# Autodesk Inventor assembly: robotface
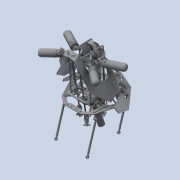
[picture p0: Inventor's stored thumbnail of the model, 180x180]
Saved by Autodesk Inventor 2020 (Build 240168000, 168)
## iProperties
Created: 2021-06-30
Part Number: robotface
Document SubType Name: Assembly
Designer: valer
Author: valer
## Documents named in this file (49)
- C:\Users\Val\Desktop\drummingrobot\design\robotface\robotface.iam
- C:\Users\Val\Desktop\drummingrobot\design\robotface\robotface-final.ipt
- C:\Users\Val\Desktop\drummingrobot\src\parts\external\HingedThreadedStandoffPart2.ipt
- C:\Users\Val\Desktop\drummingrobot\src\parts\external\HingedThreadedStandoffPart1.ipt
- C:\Users\Val\Desktop\drummingrobot\design\robotface\TongueMount.ipt
- C:\Users\Val\Desktop\drummingrobot\design\robotface\HeadMount.ipt
- C:\Users\Val\Desktop\drummingrobot\design\robotface\LinearBearing-1612-0612-0035.ipt
- C:\Users\Val\Desktop\drummingrobot\design\robotface\ClampingHub1301-0016-0012.ipt
- C:\Users\Val\Desktop\drummingrobot\design\robotface\UJoint6D\UJoint6D-Body-4003-1006-1006.ipt
- C:\Users\Val\Desktop\drummingrobot\design\robotface\UJoint6D\UJoint6D-CenterDrive-4003-1006-1006.ipt
- C:\Users\Val\Desktop\drummingrobot\design\robotface\UJoint6D\UJoint6D-Screw.ipt
- C:\Users\Val\Desktop\drummingrobot\design\robotface\SetScrewLiteHub-1308-0016-0006.ipt
- C:\Users\Val\Desktop\drummingrobot\design\robotface\ShaftD6-Short-2101-0006-0020.ipt
- C:\Users\Val\Desktop\drummingrobot\design\robotface\SetScrewHub-1300-0016-1006.ipt
- C:\Users\Val\Desktop\drummingrobot\design\robotface\ShaftD6Female-632Female.ipt
- C:\Users\Val\Desktop\drummingrobot\design\robotface\ShaftD6-2101-0006-0160.ipt
- C:\Users\Val\Desktop\drummingrobot\design\robotface\HeadTongueMount.ipt
- C:\Users\Val\Desktop\drummingrobot\design\robotface\ShaftD6-2100-0006-0250.ipt
- C:\Users\Val\Desktop\drummingrobot\design\robotface\Rod4mm.ipt
- C:\Users\Val\Desktop\drummingrobot\design\robotface\NoseBentBar.ipt
- C:\Users\Val\Desktop\drummingrobot\design\robotface\HeadTopConnector.ipt
- C:\Users\Val\Desktop\drummingrobot\design\robotface\GoTube-4103-0032-0120.ipt
- C:\Users\Val\Desktop\drummingrobot\design\robotface\UJointSq-4005-0016-0001\4005-0016-0001 Ball.ipt
- C:\Users\Val\Desktop\drummingrobot\design\robotface\UJointSq-4005-0016-0001\4005-0016-0001 Outer Shell.ipt
- C:\Users\Val\Desktop\drummingrobot\design\robotface\7417N62_INTERNALLY THREADED CONNECTING ROD.ipt
- C:\Users\Val\Desktop\drummingrobot\design\robotface\RodEndFixed-2434K495_CORROSION-RESISTANT FULLY THREADED ROD END BOLT.ipt
- C:\Users\Val\Desktop\drummingrobot\design\robotface\StandoffM4-1501-0006-0420.ipt
- C:\Users\Val\Desktop\drummingrobot\design\robotface\StandoffM4-1501-0006-0340.ipt
- C:\Users\Val\Desktop\drummingrobot\src\parts\external\Arducam.ipt
- C:\Users\Val\Desktop\drummingrobot\src\parts\external\ArducamHat.ipt
- C:\Users\Val\Desktop\drummingrobot\design\robotface\HeadEyeMount.ipt
- C:\Users\Val\Desktop\drummingrobot\design\robotface\M3-Standoff-30mm.ipt
- C:\Users\Val\Desktop\drummingrobot\design\robotface\M5-Standoff-32mm.ipt
- C:\Users\Val\Desktop\drummingrobot\src\parts\external\ArducamMirror.ipt
- C:\Users\Val\Desktop\drummingrobot\design\robotface\M1-Standoff-20mm.ipt
- C:\Users\Val\Desktop\drummingrobot\design\robotface\NoseInsideConnector.ipt
- C:\Users\Val\Desktop\drummingrobot\design\robotface\Part2^3mm U-Joint.ipt
- C:\Users\Val\Desktop\drummingrobot\design\robotface\Part1^3mm U-Joint.ipt
- C:\Users\Val\Desktop\drummingrobot\design\robotface\NoseCover.ipt
- C:\Users\Val\Desktop\drummingrobot\design\robotface\NoseCoverSmall.ipt
- C:\Users\Val\Desktop\drummingrobot\design\robotface\IRLed-FY-4006.ipt
- C:\Users\Val\Desktop\drummingrobot\design\robotface\BackEyeMountLeft.ipt
- C:\Users\Val\Desktop\drummingrobot\design\robotface\BackEyeMountRight.ipt
- C:\Users\Val\Desktop\drummingrobot\design\robotface\ShaftClamp6-6058N14.ipt
- C:\Users\Val\Desktop\drummingrobot\design\robotface\MuzzleHeadMount.ipt
- C:\Users\Val\Desktop\drummingrobot\design\robotface\ShaftD6-2100-0006-0200.ipt
- C:\Users\Val\Desktop\drummingrobot\design\robotface\MuzzleHeadConnector.ipt
- C:\Users\Val\Desktop\drummingrobot\src\parts\VacuumTubeHolder.iam
- C:\Users\Val\Desktop\drummingrobot\src\parts\FaceTubeConnector.ipt
## Components (180 placed, 48 different names)
1. robotface-final:1 — Mate:7, Mate:8, Mate:9, Mate:10, Mate:11, Mate:12, Angle:3, Mate:18, Mate:19, Mate:20, Mate:25, Mate:26, Mate:90, Mate:91, Mate:92, Mate:93, Angle:18, Angle:20, Mate:132, Mate:133, Angle:28, Mate:189, Mate:190, Angle:35, Angle:36, Mate:205, Angle:41, Mate:242, Mate:244, Mate:245, Mate:246, Mate:247, Mate:248, Mate:249, Mate:250, Mate:251, Mate:254, Mate:255, Angle:47, Mate:277, Mate:278, Mate:282, Mate:368, Mate:369, Angle:58, Mate:380, Mate:381, Mate:382, Mate:383, Mate:386, Mate:387, Mate:389, Mate:404, Mate:405, Mate:414, Mate:415, Mate:416, Mate:417, Mate:418, Mate:419, Mate:463, Mate:465, Mate:469, Mate:474
2. HingedThreadedStandoffPart2:1 — Mate:1, Mate:2, Flush:1, Angle:4, Mate:284
3. HingedThreadedStandoffPart1:1 — Mate:1, Mate:2, Mate:7, Mate:8
4. HingedThreadedStandoffPart2:2 — Mate:3, Mate:4, Mate:9, Mate:10
5. HingedThreadedStandoffPart1:2 — Mate:3, Mate:4, Flush:1
6. HingedThreadedStandoffPart2:3 — Mate:5, Mate:6, Mate:11, Mate:12, Angle:3, Mate:60, Mate:61
7. HingedThreadedStandoffPart1:3 — Mate:5, Mate:6, Angle:4
8. HingedThreadedStandoffPart2:4 — Mate:18, Mate:19, Mate:20, Mate:21, Mate:22
9. HingedThreadedStandoffPart1:4 — Mate:21, Mate:22, Mate:89
10. HingedThreadedStandoffPart2:5 — Mate:25, Mate:26
11. HingedThreadedStandoffPart1:5 — Mate:85, Mate:86
12. TongueMount:2 — Mate:278, Mate:281, Mate:283, Mate:284, Flush:24
13. HeadMount:1 — Mate:110, Mate:111, Mate:112, Flush:12, Mate:210, Mate:211, Mate:212, Mate:213, Mate:214, Mate:215, Mate:216, Mate:217, Mate:342, Mate:345, Mate:346, Mate:347, Mate:392, Mate:393, Mate:394, Mate:398, Mate:399, Mate:400
14. LinearBearing-1612-0612-0035:1 — Mate:299, Mate:300, Flush:25
15. ClampingHub1301-0016-0012:1 — Mate:115, Mate:282, Mate:300, Flush:25
16. ShaftD6-2100-0006-0250:1 — Mate:298, Angle:52, Flush:23, Angle:54, Mate:299, Mate:311, Angle:55, Flush:26
17. SetScrewLiteHub-1308-0016-0006:1 — Mate:65, Mate:67, Mate:281, Angle:53, Flush:24
18. HingedThreadedStandoffPart2:6 — Mate:60, Mate:61, Mate:283
19. ShaftD6-Short-2101-0006-0020:1 — Mate:65, Mate:67, Angle:51, Mate:297, Flush:22
20. ShaftD6-2101-0006-0160:2 — Mate:87, Angle:16
21. ShaftD6-2101-0006-0160:3
22. SetScrewHub-1300-0016-1006:1 — Mate:114
23. SetScrewHub-1300-0016-1006:2 — Mate:113
24. ShaftD6Female-632Female:1 — Mate:85, Mate:86
25. ShaftD6Female-632Female:2 — Mate:87, Mate:89, Angle:16
26. HingedThreadedStandoffPart2:9 — Mate:92, Mate:93, Mate:96, Mate:97
27. HingedThreadedStandoffPart2:10 — Mate:90, Mate:91, Mate:94, Mate:95
28. HingedThreadedStandoffPart2:11 — Mate:94, Mate:95, Mate:98, Mate:99
29. HingedThreadedStandoffPart2:12 — Mate:96, Mate:97, Mate:100, Mate:101
30. ShaftD6Female-632Female:3 — Mate:98, Mate:99, Mate:102, Angle:17, Mate:103, Angle:18
31. ShaftD6Female-632Female:4 — Mate:100, Mate:101, Mate:104, Angle:19, Angle:20, Mate:105
32. ShaftD6-2101-0006-0160:4 — Mate:102, Angle:17, Mate:103, Mate:106, Angle:21
33. ShaftD6-2101-0006-0160:5 — Mate:104, Angle:19, Mate:105, Mate:107, Angle:22
34. SetScrewHub-1300-0016-1006:3 — Mate:106, Angle:21, Mate:116
35. SetScrewHub-1300-0016-1006:4 — Mate:107, Angle:22, Mate:117
36. HeadTongueMount:1 — Mate:110, Mate:111, Mate:112, Mate:113, Mate:114, Mate:115, Mate:116, Mate:117, Mate:204, Angle:39, Flush:15, Angle:54, Mate:431
37. Rod4mm:1 — Mate:132
38. Rod4mm:2 — Mate:133
39. SetScrewLiteHub-1308-0016-0006:2 — Mate:151, Flush:5, Mate:153, Angle:26, Mate:242, Mate:370, Mate:371
40. UJoint6D-Body-4003-1006-1006:5 — Mate:154, Angle:27, Flush:6, Angle:28
41. UJoint6D-CenterDrive-4003-1006-1006:3
42. UJoint6D-Screw:11
43. UJoint6D-Body-4003-1006-1006:6 — Mate:152, Angle:25, Mate:153, Angle:26
44. UJoint6D-Screw:12
45. UJoint6D-Screw:13
46. UJoint6D-Screw:14
47. ShaftD6-Short-2101-0006-0020:2 — Mate:151, Flush:5, Mate:152, Angle:25
48. ShaftD6-2100-0006-0250:2 — Mate:154, Angle:27, Flush:6, Mate:167, Angle:29, Flush:7
49. UJoint6D-Body-4003-1006-1006:7 — Mate:184, Angle:32, Flush:9, Mate:185, Angle:38
50. UJoint6D-CenterDrive-4003-1006-1006:4
51. UJoint6D-Screw:15
52. UJoint6D-Body-4003-1006-1006:8 — Mate:167, Angle:29, Flush:7
53. UJoint6D-Screw:16
54. UJoint6D-Screw:17
55. UJoint6D-Screw:18
56. SetScrewLiteHub-1308-0016-0006:3 — Mate:185, Mate:186, Angle:38
57. ShaftD6-Short-2101-0006-0020:3 — Mate:184, Angle:32, Flush:9, Mate:186
58. ShaftD6-Short-2101-0006-0020:4 — Mate:312, Angle:56, Flush:27, Mate:313, Flush:28
59. NoseBentBar:1 — Mate:189, Angle:36, Flush:13, Flush:14
60. NoseBentBar:2 — Mate:190, Angle:35, Flush:13
61. HeadTopConnector:1 — Flush:12, Flush:14
62. GoTube-4103-0032-0120:1 — Mate:201, Mate:202, Mate:203
63. 4005-0016-0001 Ball:1 — Mate:197, Mate:198, Mate:199, Mate:200
64. 4005-0016-0001 Outer Shell:1 — Mate:197, Mate:198, Mate:204, Angle:39, Flush:15, Mate:205
65. 4005-0016-0001 Outer Shell:2 — Mate:199, Mate:200, Mate:201, Mate:202, Mate:203
66. 7417N62_INTERNALLY THREADED CONNECTING ROD:1 — Mate:218, Mate:219, Mate:220, Mate:222
67. RodEndFixed-2434K495_CORROSION-RESISTANT FULLY THREADED ROD END BOLT:1 — Mate:210, Mate:211, Angle:40, Angle:41, Angle:42, Mate:221, Mate:223
68. RodEndFixed-2434K495_CORROSION-RESISTANT FULLY THREADED ROD END BOLT:2 — Mate:212, Mate:213, Angle:40, Mate:228, Mate:229
69. RodEndFixed-2434K495_CORROSION-RESISTANT FULLY THREADED ROD END BOLT:3 — Mate:214, Mate:215, Angle:42, Angle:43, Mate:240, Mate:241
70. RodEndFixed-2434K495_CORROSION-RESISTANT FULLY THREADED ROD END BOLT:4 — Mate:216, Mate:217, Angle:43, Mate:234, Mate:235
71. RodEndFixed-2434K495_CORROSION-RESISTANT FULLY THREADED ROD END BOLT:5 — Mate:218, Mate:220, Mate:221, Mate:223
72. RodEndFixed-2434K495_CORROSION-RESISTANT FULLY THREADED ROD END BOLT:6 — Mate:219, Mate:222, Angle:44, Angle:46
73. 7417N62_INTERNALLY THREADED CONNECTING ROD:2
74. RodEndFixed-2434K495_CORROSION-RESISTANT FULLY THREADED ROD END BOLT:7 — Mate:228, Mate:229
75. RodEndFixed-2434K495_CORROSION-RESISTANT FULLY THREADED ROD END BOLT:8 — Angle:44, Angle:45
76. 7417N62_INTERNALLY THREADED CONNECTING ROD:3
77. RodEndFixed-2434K495_CORROSION-RESISTANT FULLY THREADED ROD END BOLT:9 — Mate:234, Mate:235
78. RodEndFixed-2434K495_CORROSION-RESISTANT FULLY THREADED ROD END BOLT:10 — Angle:45
79. 7417N62_INTERNALLY THREADED CONNECTING ROD:4
80. RodEndFixed-2434K495_CORROSION-RESISTANT FULLY THREADED ROD END BOLT:11 — Mate:240, Mate:241
81. RodEndFixed-2434K495_CORROSION-RESISTANT FULLY THREADED ROD END BOLT:12 — Angle:46
82. StandoffM4-1501-0006-0420:1 — Mate:244, Mate:245
83. StandoffM4-1501-0006-0420:2 — Mate:246, Mate:247
84. StandoffM4-1501-0006-0340:1 — Mate:248, Mate:249
85. StandoffM4-1501-0006-0340:2 — Mate:250, Mate:251
86. HingedThreadedStandoffPart2:13 — Mate:256, Mate:257
87. HingedThreadedStandoffPart1:6 — Mate:254, Mate:255, Angle:47
88. ShaftD6Female-632Female:5 — Mate:256, Mate:257, Mate:273, Angle:50, Mate:274
89. ShaftD6-2100-0006-0250:3 — Mate:273, Angle:50, Mate:274
90. UJoint6D-Body-4003-1006-1006:9
91. UJoint6D-CenterDrive-4003-1006-1006:5
92. UJoint6D-Screw:19
93. UJoint6D-Body-4003-1006-1006:10
94. UJoint6D-Screw:20
95. UJoint6D-Screw:21
96. UJoint6D-Screw:22
97. SetScrewLiteHub-1308-0016-0006:5
98. ShaftD6-Short-2101-0006-0020:5
99. ArducamHat:1 — Mate:314, Mate:316, Mate:317, Mate:318, Mate:319
100. Arducam:2 — Mate:350, Mate:351, Mate:352, Mate:354, Mate:356, Mate:364, Mate:390
101. HeadEyeMount:1 — Mate:277, Mate:315, Mate:320, Mate:341, Mate:343, Mate:344, Mate:348, Mate:349, Mate:350, Mate:351, Mate:353, Mate:355, Mate:357, Mate:359, Mate:360, Mate:362, Mate:365, Mate:367
102. UJoint6D-Body-4003-1006-1006:11 — Mate:298, Angle:52, Flush:23
103. UJoint6D-CenterDrive-4003-1006-1006:6
104. UJoint6D-Screw:23
105. UJoint6D-Body-4003-1006-1006:12 — Angle:51, Mate:297, Flush:22, Angle:53
106. UJoint6D-Screw:24
107. UJoint6D-Screw:25
108. UJoint6D-Screw:26
109. UJoint6D-Body-4003-1006-1006:13 — Mate:312, Angle:56, Flush:27, Angle:57
110. UJoint6D-CenterDrive-4003-1006-1006:7
111. UJoint6D-Body-4003-1006-1006:14 — Mate:311, Angle:55, Flush:26
112. UJoint6D-Screw:27
113. UJoint6D-Screw:28
114. UJoint6D-Screw:29
115. SetScrewLiteHub-1308-0016-0006:6 — Mate:313, Angle:57, Flush:28
116. M3-Standoff-30mm:1 — Mate:314, Mate:315, Mate:316
117. M3-Standoff-30mm:2 — Mate:317, Mate:318
118. M3-Standoff-30mm:3 — Mate:319, Mate:320
119. M5-Standoff-32mm:1 — Mate:341, Mate:342, Mate:343
120. M5-Standoff-32mm:2 — Mate:344, Mate:345
121. M5-Standoff-32mm:3 — Mate:346, Mate:349
122. M5-Standoff-32mm:4 — Mate:347, Mate:348
123. ArducamMirror:1 — Mate:358, Mate:361, Mate:363, Mate:366, Mate:391
124. M1-Standoff-20mm:1 — Mate:352, Mate:353
125. M1-Standoff-20mm:2 — Mate:354, Mate:355, Mate:364
126. M1-Standoff-20mm:3 — Mate:356, Mate:357
127. M1-Standoff-20mm:4 — Mate:358, Mate:359, Mate:360
128. M1-Standoff-20mm:5 — Mate:361, Mate:362, Mate:363, Mate:365
129. M1-Standoff-20mm:6 — Mate:366, Mate:367
130. NoseInsideConnector:1 — Mate:368, Mate:369, Angle:58, Mate:370, Mate:371, Mate:384, Mate:385
131. Part2^3mm U-Joint:1 — Mate:372, Mate:373, Mate:374, Mate:375
132. Part1^3mm U-Joint:1 — Mate:372, Mate:373, Mate:385
133. Part1^3mm U-Joint:2 — Mate:374, Mate:375, Mate:380, Mate:381
134. Part2^3mm U-Joint:2
135. Part1^3mm U-Joint:3 — Mate:384
136. Part1^3mm U-Joint:4 — Mate:382, Mate:383
137. NoseCover:1 — Mate:386, Mate:387, Flush:29, Mate:388
138. NoseCoverSmall:1 — Flush:29, Mate:388, Mate:389
139. IRLed-FY-4006:1 — Mate:391
140. IRLed-FY-4006:2 — Mate:390
141. IRLed-FY-4006:3 — Mate:395, Mate:396, Mate:397
142. BackEyeMountRight:1 — Mate:398, Mate:399, Mate:400, Mate:401, Mate:402, Mate:403
143. BackEyeMountLeft:1 — Mate:392, Mate:393, Mate:394, Mate:395, Mate:396, Mate:397
144. IRLed-FY-4006:4 — Mate:401, Mate:402, Mate:403
145. ShaftD6-2100-0006-0200:1 — Mate:432, Mate:436
146. ShaftClamp6-6058N14:1 — Mate:404, Mate:405
147. ShaftD6-2100-0006-0200:2 — Mate:441, Mate:443, Mate:458
148. ShaftClamp6-6058N14:2 — Mate:464
149. ShaftD6-2100-0006-0200:3 — Mate:445, Mate:447, Mate:466
150. ShaftClamp6-6058N14:3
151. ShaftClamp6-6058N14:4 — Mate:414, Mate:415
152. ShaftClamp6-6058N14:5 — Mate:416, Mate:417
153. ShaftD6-2100-0006-0200:4 — Mate:437, Mate:439
154. ShaftClamp6-6058N14:6 — Mate:418, Mate:419
155. ShaftD6-2100-0006-0200:5 — Mate:449, Mate:451, Mate:475
156. ShaftClamp6-6058N14:7 — Mate:476
157. ShaftD6-2100-0006-0200:6 — Mate:453, Mate:455, Mate:470
158. ShaftClamp6-6058N14:8 — Mate:471
159. MuzzleHeadMount:1 — Mate:428, Mate:429, Mate:430, Mate:434, Mate:435, Mate:438, Mate:440, Mate:442, Mate:444, Mate:446, Mate:448, Mate:450, Mate:452, Mate:454, Mate:456
160. MuzzleHeadConnector:1 — Mate:428, Mate:429, Mate:430, Mate:431
161. ShaftClamp6-6058N14:9 — Mate:432, Mate:434
162. ShaftClamp6-6058N14:10 — Mate:435, Mate:436
163. ShaftClamp6-6058N14:12 — Mate:437, Mate:438
164. ShaftClamp6-6058N14:13 — Mate:439, Mate:440
165. ShaftClamp6-6058N14:14 — Mate:441, Mate:442
166. ShaftClamp6-6058N14:15 — Mate:443, Mate:444
167. ShaftClamp6-6058N14:16 — Mate:445, Mate:446
168. ShaftClamp6-6058N14:17 — Mate:447, Mate:448
169. ShaftClamp6-6058N14:18 — Mate:449, Mate:450
170. ShaftClamp6-6058N14:19 — Mate:451, Mate:452
171. ShaftClamp6-6058N14:20 — Mate:453, Mate:454
172. ShaftClamp6-6058N14:21 — Mate:455, Mate:456
173. VacuumTubeHolder:1 [sub-assembly] — Mate:467, Mate:468
174. VacuumTubeHolder:2 [sub-assembly] — Mate:461, Mate:462
175. VacuumTubeHolder:3 [sub-assembly] — Mate:477, Mate:478
176. VacuumTubeHolder:4 [sub-assembly] — Mate:472, Mate:473
177. BackSideConnector:1 — Mate:458, Mate:461, Mate:462, Mate:463, Mate:464
178. BackSideConnector:2 — Mate:465, Mate:466, Mate:467, Mate:468
179. BackSideConnector:3 — Mate:469, Mate:470, Mate:471, Mate:472, Mate:473
180. BackSideConnector:4 — Mate:474, Mate:475, Mate:476, Mate:477, Mate:478
## Relationships (411: Mate 342, Angle 45, Flush 24)
- Mate:1: HingedThreadedStandoffPart2:1 ↔ HingedThreadedStandoffPart1:1
- Mate:2: HingedThreadedStandoffPart2:1 ↔ HingedThreadedStandoffPart1:1
- Mate:3: HingedThreadedStandoffPart2:2 ↔ HingedThreadedStandoffPart1:2
- Mate:4: HingedThreadedStandoffPart2:2 ↔ HingedThreadedStandoffPart1:2
- Mate:5: HingedThreadedStandoffPart2:3 ↔ HingedThreadedStandoffPart1:3
- Mate:6: HingedThreadedStandoffPart2:3 ↔ HingedThreadedStandoffPart1:3
- Mate:7: robotface-final:1 ↔ HingedThreadedStandoffPart1:1
- Mate:8: robotface-final:1 ↔ HingedThreadedStandoffPart1:1
- Mate:9: robotface-final:1 ↔ HingedThreadedStandoffPart2:2
- Mate:10: robotface-final:1 ↔ HingedThreadedStandoffPart2:2
- Mate:11: robotface-final:1 ↔ HingedThreadedStandoffPart2:3
- Mate:12: robotface-final:1 ↔ HingedThreadedStandoffPart2:3
- Angle:3 (0 deg): robotface-final:1 ↔ HingedThreadedStandoffPart2:3
- Mate:18: robotface-final:1 ↔ HingedThreadedStandoffPart2:4
- Mate:19: robotface-final:1 ↔ HingedThreadedStandoffPart2:4
- Mate:20: robotface-final:1 ↔ HingedThreadedStandoffPart2:4
- Mate:21: HingedThreadedStandoffPart2:4 ↔ HingedThreadedStandoffPart1:4
- Mate:22: HingedThreadedStandoffPart2:4 ↔ HingedThreadedStandoffPart1:4
- [Mate]: HingedThreadedStandoffPart2:5 ↔ HingedThreadedStandoffPart1:5
- [Mate]: HingedThreadedStandoffPart2:5 ↔ HingedThreadedStandoffPart1:5
- Mate:25: robotface-final:1 ↔ HingedThreadedStandoffPart2:5
- Mate:26: robotface-final:1 ↔ HingedThreadedStandoffPart2:5
- Flush:1: HingedThreadedStandoffPart2:1 ↔ HingedThreadedStandoffPart1:2
- Angle:4 (0 deg): HingedThreadedStandoffPart2:1 ↔ HingedThreadedStandoffPart1:3
- Mate:60: HingedThreadedStandoffPart2:3 ↔ HingedThreadedStandoffPart2:6
- Mate:61: HingedThreadedStandoffPart2:3 ↔ HingedThreadedStandoffPart2:6
- Mate:65: SetScrewLiteHub-1308-0016-0006:1 ↔ ShaftD6-Short-2101-0006-0020:1
- Mate:67 (-7 mm): SetScrewLiteHub-1308-0016-0006:1 ↔ ShaftD6-Short-2101-0006-0020:1
- [Mate]: HingedThreadedStandoffPart1:4 ↔ ShaftD6-2101-0006-0160:2
- [Angle] (0 deg): HeadMount:1 ↔ ShaftD6-2101-0006-0160:2
- [Mate]: HingedThreadedStandoffPart1:5 ↔ ShaftD6-2101-0006-0160:3
- [Angle] (0 deg): HeadMount:1 ↔ ShaftD6-2101-0006-0160:3
- [Mate]: ShaftD6-2101-0006-0160:2 ↔ SetScrewHub-1300-0016-1006:1
- [Mate]: ShaftD6-2101-0006-0160:3 ↔ SetScrewHub-1300-0016-1006:2
- [Angle] (0 deg): ShaftD6-2101-0006-0160:2 ↔ SetScrewHub-1300-0016-1006:1
- [Angle] (0 deg): ShaftD6-2101-0006-0160:3 ↔ SetScrewHub-1300-0016-1006:2
- [Angle] (0 deg): robotface-final:1 ↔ ShaftD6-2101-0006-0160:2
- [Angle] (0 deg): robotface-final:1 ↔ ShaftD6-2101-0006-0160:3
- [Mate]: ShaftD6-2101-0006-0160:3 ↔ ShaftD6Female-632Female:1
- [Angle] (0 deg): ShaftD6-2101-0006-0160:3 ↔ ShaftD6Female-632Female:1
- [Mate]: ShaftD6-2101-0006-0160:3 ↔ ShaftD6Female-632Female:1
- Mate:85: HingedThreadedStandoffPart1:5 ↔ ShaftD6Female-632Female:1
- Mate:86: HingedThreadedStandoffPart1:5 ↔ ShaftD6Female-632Female:1
- Mate:87: ShaftD6-2101-0006-0160:2 ↔ ShaftD6Female-632Female:2
- Mate:89: HingedThreadedStandoffPart1:4 ↔ ShaftD6Female-632Female:2
- Angle:16 (0 deg): ShaftD6-2101-0006-0160:2 ↔ ShaftD6Female-632Female:2
- Mate:90: robotface-final:1 ↔ HingedThreadedStandoffPart2:10
- Mate:91: robotface-final:1 ↔ HingedThreadedStandoffPart2:10
- Mate:92: robotface-final:1 ↔ HingedThreadedStandoffPart2:9
- Mate:93: robotface-final:1 ↔ HingedThreadedStandoffPart2:9
- Mate:94: HingedThreadedStandoffPart2:10 ↔ HingedThreadedStandoffPart2:11
- Mate:95: HingedThreadedStandoffPart2:10 ↔ HingedThreadedStandoffPart2:11
- Mate:96: HingedThreadedStandoffPart2:9 ↔ HingedThreadedStandoffPart2:12
- Mate:97: HingedThreadedStandoffPart2:9 ↔ HingedThreadedStandoffPart2:12
- Mate:98: HingedThreadedStandoffPart2:11 ↔ ShaftD6Female-632Female:3
- Mate:99: HingedThreadedStandoffPart2:11 ↔ ShaftD6Female-632Female:3
- Mate:100: HingedThreadedStandoffPart2:12 ↔ ShaftD6Female-632Female:4
- Mate:101: HingedThreadedStandoffPart2:12 ↔ ShaftD6Female-632Female:4
- Mate:102: ShaftD6Female-632Female:3 ↔ ShaftD6-2101-0006-0160:4
- Angle:17 (0 deg): ShaftD6Female-632Female:3 ↔ ShaftD6-2101-0006-0160:4
- Mate:103: ShaftD6Female-632Female:3 ↔ ShaftD6-2101-0006-0160:4
- Angle:18 (180 deg): robotface-final:1 ↔ ShaftD6Female-632Female:3
- Mate:104: ShaftD6Female-632Female:4 ↔ ShaftD6-2101-0006-0160:5
- Angle:19 (0 deg): ShaftD6Female-632Female:4 ↔ ShaftD6-2101-0006-0160:5
- Angle:20 (180 deg): robotface-final:1 ↔ ShaftD6Female-632Female:4
- Mate:105: ShaftD6Female-632Female:4 ↔ ShaftD6-2101-0006-0160:5
- Mate:106: ShaftD6-2101-0006-0160:4 ↔ SetScrewHub-1300-0016-1006:3
- Angle:21 (180 deg): ShaftD6-2101-0006-0160:4 ↔ SetScrewHub-1300-0016-1006:3
- Mate:107: ShaftD6-2101-0006-0160:5 ↔ SetScrewHub-1300-0016-1006:4
- Angle:22 (180 deg): ShaftD6-2101-0006-0160:5 ↔ SetScrewHub-1300-0016-1006:4
- Mate:110: HeadMount:1 ↔ HeadTongueMount:1
- Mate:111: HeadMount:1 ↔ HeadTongueMount:1
- Mate:112: HeadMount:1 ↔ HeadTongueMount:1
- Mate:113: SetScrewHub-1300-0016-1006:2 ↔ HeadTongueMount:1
- Mate:114: SetScrewHub-1300-0016-1006:1 ↔ HeadTongueMount:1
- Mate:115: ClampingHub1301-0016-0012:1 ↔ HeadTongueMount:1
- Mate:116: SetScrewHub-1300-0016-1006:3 ↔ HeadTongueMount:1
- Mate:117: SetScrewHub-1300-0016-1006:4 ↔ HeadTongueMount:1
- Mate:132: robotface-final:1 ↔ Rod4mm:1
- Mate:133: robotface-final:1 ↔ Rod4mm:2
- [Mate]: UJoint6D-CenterDrive-4003-1006-1006:3 ↔ UJoint6D-Body-4003-1006-1006:6
- [Mate]: UJoint6D-CenterDrive-4003-1006-1006:3 ↔ UJoint6D-Body-4003-1006-1006:6
- [Mate]: UJoint6D-Body-4003-1006-1006:5 ↔ UJoint6D-CenterDrive-4003-1006-1006:3
- [Mate]: UJoint6D-Body-4003-1006-1006:5 ↔ UJoint6D-CenterDrive-4003-1006-1006:3
- [Mate]: UJoint6D-Body-4003-1006-1006:5 ↔ UJoint6D-Screw:11
- [Mate]: UJoint6D-Body-4003-1006-1006:5 ↔ UJoint6D-Screw:11
- [Mate]: UJoint6D-Body-4003-1006-1006:5 ↔ UJoint6D-Screw:13
- [Mate]: UJoint6D-Body-4003-1006-1006:5 ↔ UJoint6D-Screw:13
- [Mate]: UJoint6D-Body-4003-1006-1006:6 ↔ UJoint6D-Screw:12
- [Mate]: UJoint6D-Body-4003-1006-1006:6 ↔ UJoint6D-Screw:12
- [Mate]: UJoint6D-Body-4003-1006-1006:6 ↔ UJoint6D-Screw:14
- [Mate]: UJoint6D-Body-4003-1006-1006:6 ↔ UJoint6D-Screw:14
- Mate:151: SetScrewLiteHub-1308-0016-0006:2 ↔ ShaftD6-Short-2101-0006-0020:2
- Flush:5: SetScrewLiteHub-1308-0016-0006:2 ↔ ShaftD6-Short-2101-0006-0020:2
- Mate:152: UJoint6D-Body-4003-1006-1006:6 ↔ ShaftD6-Short-2101-0006-0020:2
- Angle:25 (180 deg): UJoint6D-Body-4003-1006-1006:6 ↔ ShaftD6-Short-2101-0006-0020:2
- Mate:153: SetScrewLiteHub-1308-0016-0006:2 ↔ UJoint6D-Body-4003-1006-1006:6
- Angle:26 (0 deg): SetScrewLiteHub-1308-0016-0006:2 ↔ UJoint6D-Body-4003-1006-1006:6
- Mate:154: UJoint6D-Body-4003-1006-1006:5 ↔ ShaftD6-2100-0006-0250:2
- Angle:27 (180 deg): UJoint6D-Body-4003-1006-1006:5 ↔ ShaftD6-2100-0006-0250:2
- Flush:6: UJoint6D-Body-4003-1006-1006:5 ↔ ShaftD6-2100-0006-0250:2
- Angle:28 (0 deg): robotface-final:1 ↔ UJoint6D-Body-4003-1006-1006:5
- [Mate]: UJoint6D-CenterDrive-4003-1006-1006:4 ↔ UJoint6D-Body-4003-1006-1006:8
- [Mate]: UJoint6D-CenterDrive-4003-1006-1006:4 ↔ UJoint6D-Body-4003-1006-1006:8
- [Mate]: UJoint6D-Body-4003-1006-1006:7 ↔ UJoint6D-CenterDrive-4003-1006-1006:4
- [Mate]: UJoint6D-Body-4003-1006-1006:7 ↔ UJoint6D-CenterDrive-4003-1006-1006:4
- [Mate]: UJoint6D-Body-4003-1006-1006:7 ↔ UJoint6D-Screw:15
- [Mate]: UJoint6D-Body-4003-1006-1006:7 ↔ UJoint6D-Screw:15
- [Mate]: UJoint6D-Body-4003-1006-1006:7 ↔ UJoint6D-Screw:17
- [Mate]: UJoint6D-Body-4003-1006-1006:7 ↔ UJoint6D-Screw:17
- [Mate]: UJoint6D-Body-4003-1006-1006:8 ↔ UJoint6D-Screw:16
- [Mate]: UJoint6D-Body-4003-1006-1006:8 ↔ UJoint6D-Screw:16
- [Mate]: UJoint6D-Body-4003-1006-1006:8 ↔ UJoint6D-Screw:18
- [Mate]: UJoint6D-Body-4003-1006-1006:8 ↔ UJoint6D-Screw:18
- Mate:167: ShaftD6-2100-0006-0250:2 ↔ UJoint6D-Body-4003-1006-1006:8
- Angle:29 (180 deg): ShaftD6-2100-0006-0250:2 ↔ UJoint6D-Body-4003-1006-1006:8
- Flush:7: ShaftD6-2100-0006-0250:2 ↔ UJoint6D-Body-4003-1006-1006:8
- Mate:184: UJoint6D-Body-4003-1006-1006:7 ↔ ShaftD6-Short-2101-0006-0020:3
- Angle:32 (0 deg): UJoint6D-Body-4003-1006-1006:7 ↔ ShaftD6-Short-2101-0006-0020:3
- Flush:9: UJoint6D-Body-4003-1006-1006:7 ↔ ShaftD6-Short-2101-0006-0020:3
- Mate:185: UJoint6D-Body-4003-1006-1006:7 ↔ SetScrewLiteHub-1308-0016-0006:3
- Mate:186: SetScrewLiteHub-1308-0016-0006:3 ↔ ShaftD6-Short-2101-0006-0020:3
- Mate:189: robotface-final:1 ↔ NoseBentBar:1
- Mate:190: robotface-final:1 ↔ NoseBentBar:2
- Flush:12: HeadMount:1 ↔ HeadTopConnector:1
- Angle:35 (0 deg): robotface-final:1 ↔ NoseBentBar:2
- Angle:36 (0 deg): robotface-final:1 ↔ NoseBentBar:1
- Flush:13: NoseBentBar:1 ↔ NoseBentBar:2
- Flush:14: NoseBentBar:1 ↔ HeadTopConnector:1
- Angle:38 (0 deg): UJoint6D-Body-4003-1006-1006:7 ↔ SetScrewLiteHub-1308-0016-0006:3
- Mate:197: 4005-0016-0001 Ball:1 ↔ 4005-0016-0001 Outer Shell:1
- Mate:198: 4005-0016-0001 Ball:1 ↔ 4005-0016-0001 Outer Shell:1
- Mate:199: 4005-0016-0001 Ball:1 ↔ 4005-0016-0001 Outer Shell:2
- Mate:200: 4005-0016-0001 Ball:1 ↔ 4005-0016-0001 Outer Shell:2
- Mate:201: GoTube-4103-0032-0120:1 ↔ 4005-0016-0001 Outer Shell:2
- Mate:202: GoTube-4103-0032-0120:1 ↔ 4005-0016-0001 Outer Shell:2
- Mate:203: GoTube-4103-0032-0120:1 ↔ 4005-0016-0001 Outer Shell:2
- Mate:204: HeadTongueMount:1 ↔ 4005-0016-0001 Outer Shell:1
- Angle:39 (0 deg): HeadTongueMount:1 ↔ 4005-0016-0001 Outer Shell:1
- Flush:15: HeadTongueMount:1 ↔ 4005-0016-0001 Outer Shell:1
- Mate:205: robotface-final:1 ↔ 4005-0016-0001 Outer Shell:1
- Mate:210: HeadMount:1 ↔ RodEndFixed-2434K495_CORROSION-RESISTANT FULLY THREADED ROD END BOLT:1
- Mate:211 (-17.78 mm): HeadMount:1 ↔ RodEndFixed-2434K495_CORROSION-RESISTANT FULLY THREADED ROD END BOLT:1
- Mate:212: HeadMount:1 ↔ RodEndFixed-2434K495_CORROSION-RESISTANT FULLY THREADED ROD END BOLT:2
- Mate:213 (-17.78 mm): HeadMount:1 ↔ RodEndFixed-2434K495_CORROSION-RESISTANT FULLY THREADED ROD END BOLT:2
- Angle:40 (0 deg): RodEndFixed-2434K495_CORROSION-RESISTANT FULLY THREADED ROD END BOLT:1 ↔ RodEndFixed-2434K495_CORROSION-RESISTANT FULLY THREADED ROD END BOLT:2
- Angle:41 (0 deg): robotface-final:1 ↔ RodEndFixed-2434K495_CORROSION-RESISTANT FULLY THREADED ROD END BOLT:1
- Mate:214: HeadMount:1 ↔ RodEndFixed-2434K495_CORROSION-RESISTANT FULLY THREADED ROD END BOLT:3
- Mate:215 (-17.78 mm): HeadMount:1 ↔ RodEndFixed-2434K495_CORROSION-RESISTANT FULLY THREADED ROD END BOLT:3
- Angle:42 (0 deg): RodEndFixed-2434K495_CORROSION-RESISTANT FULLY THREADED ROD END BOLT:1 ↔ RodEndFixed-2434K495_CORROSION-RESISTANT FULLY THREADED ROD END BOLT:3
- Mate:216: HeadMount:1 ↔ RodEndFixed-2434K495_CORROSION-RESISTANT FULLY THREADED ROD END BOLT:4
- Mate:217 (-17.78 mm): HeadMount:1 ↔ RodEndFixed-2434K495_CORROSION-RESISTANT FULLY THREADED ROD END BOLT:4
- Angle:43 (0 deg): RodEndFixed-2434K495_CORROSION-RESISTANT FULLY THREADED ROD END BOLT:3 ↔ RodEndFixed-2434K495_CORROSION-RESISTANT FULLY THREADED ROD END BOLT:4
- Mate:218: 7417N62_INTERNALLY THREADED CONNECTING ROD:1 ↔ RodEndFixed-2434K495_CORROSION-RESISTANT FULLY THREADED ROD END BOLT:5
- Mate:219: 7417N62_INTERNALLY THREADED CONNECTING ROD:1 ↔ RodEndFixed-2434K495_CORROSION-RESISTANT FULLY THREADED ROD END BOLT:6
- Mate:220: 7417N62_INTERNALLY THREADED CONNECTING ROD:1 ↔ RodEndFixed-2434K495_CORROSION-RESISTANT FULLY THREADED ROD END BOLT:5
- Mate:221: RodEndFixed-2434K495_CORROSION-RESISTANT FULLY THREADED ROD END BOLT:1 ↔ RodEndFixed-2434K495_CORROSION-RESISTANT FULLY THREADED ROD END BOLT:5
- Mate:222: 7417N62_INTERNALLY THREADED CONNECTING ROD:1 ↔ RodEndFixed-2434K495_CORROSION-RESISTANT FULLY THREADED ROD END BOLT:6
- Mate:223: RodEndFixed-2434K495_CORROSION-RESISTANT FULLY THREADED ROD END BOLT:1 ↔ RodEndFixed-2434K495_CORROSION-RESISTANT FULLY THREADED ROD END BOLT:5
- [Mate]: 7417N62_INTERNALLY THREADED CONNECTING ROD:2 ↔ RodEndFixed-2434K495_CORROSION-RESISTANT FULLY THREADED ROD END BOLT:7
- [Mate]: 7417N62_INTERNALLY THREADED CONNECTING ROD:2 ↔ RodEndFixed-2434K495_CORROSION-RESISTANT FULLY THREADED ROD END BOLT:8
- [Mate]: 7417N62_INTERNALLY THREADED CONNECTING ROD:2 ↔ RodEndFixed-2434K495_CORROSION-RESISTANT FULLY THREADED ROD END BOLT:7
- [Mate]: 7417N62_INTERNALLY THREADED CONNECTING ROD:2 ↔ RodEndFixed-2434K495_CORROSION-RESISTANT FULLY THREADED ROD END BOLT:8
- Mate:228: RodEndFixed-2434K495_CORROSION-RESISTANT FULLY THREADED ROD END BOLT:2 ↔ RodEndFixed-2434K495_CORROSION-RESISTANT FULLY THREADED ROD END BOLT:7
- Mate:229: RodEndFixed-2434K495_CORROSION-RESISTANT FULLY THREADED ROD END BOLT:2 ↔ RodEndFixed-2434K495_CORROSION-RESISTANT FULLY THREADED ROD END BOLT:7
- Angle:44 (0 deg): RodEndFixed-2434K495_CORROSION-RESISTANT FULLY THREADED ROD END BOLT:6 ↔ RodEndFixed-2434K495_CORROSION-RESISTANT FULLY THREADED ROD END BOLT:8
- [Mate]: 7417N62_INTERNALLY THREADED CONNECTING ROD:3 ↔ RodEndFixed-2434K495_CORROSION-RESISTANT FULLY THREADED ROD END BOLT:9
- [Mate]: 7417N62_INTERNALLY THREADED CONNECTING ROD:3 ↔ RodEndFixed-2434K495_CORROSION-RESISTANT FULLY THREADED ROD END BOLT:10
- [Mate]: 7417N62_INTERNALLY THREADED CONNECTING ROD:3 ↔ RodEndFixed-2434K495_CORROSION-RESISTANT FULLY THREADED ROD END BOLT:9
- [Mate]: 7417N62_INTERNALLY THREADED CONNECTING ROD:3 ↔ RodEndFixed-2434K495_CORROSION-RESISTANT FULLY THREADED ROD END BOLT:10
- Mate:234: RodEndFixed-2434K495_CORROSION-RESISTANT FULLY THREADED ROD END BOLT:4 ↔ RodEndFixed-2434K495_CORROSION-RESISTANT FULLY THREADED ROD END BOLT:9
- Mate:235: RodEndFixed-2434K495_CORROSION-RESISTANT FULLY THREADED ROD END BOLT:4 ↔ RodEndFixed-2434K495_CORROSION-RESISTANT FULLY THREADED ROD END BOLT:9
- Angle:45 (0 deg): RodEndFixed-2434K495_CORROSION-RESISTANT FULLY THREADED ROD END BOLT:8 ↔ RodEndFixed-2434K495_CORROSION-RESISTANT FULLY THREADED ROD END BOLT:10
- [Mate]: 7417N62_INTERNALLY THREADED CONNECTING ROD:4 ↔ RodEndFixed-2434K495_CORROSION-RESISTANT FULLY THREADED ROD END BOLT:11
- [Mate]: 7417N62_INTERNALLY THREADED CONNECTING ROD:4 ↔ RodEndFixed-2434K495_CORROSION-RESISTANT FULLY THREADED ROD END BOLT:12
- [Mate]: 7417N62_INTERNALLY THREADED CONNECTING ROD:4 ↔ RodEndFixed-2434K495_CORROSION-RESISTANT FULLY THREADED ROD END BOLT:11
- [Mate]: 7417N62_INTERNALLY THREADED CONNECTING ROD:4 ↔ RodEndFixed-2434K495_CORROSION-RESISTANT FULLY THREADED ROD END BOLT:12
- Mate:240: RodEndFixed-2434K495_CORROSION-RESISTANT FULLY THREADED ROD END BOLT:3 ↔ RodEndFixed-2434K495_CORROSION-RESISTANT FULLY THREADED ROD END BOLT:11
- Mate:241: RodEndFixed-2434K495_CORROSION-RESISTANT FULLY THREADED ROD END BOLT:3 ↔ RodEndFixed-2434K495_CORROSION-RESISTANT FULLY THREADED ROD END BOLT:11
- Angle:46 (0 deg): RodEndFixed-2434K495_CORROSION-RESISTANT FULLY THREADED ROD END BOLT:6 ↔ RodEndFixed-2434K495_CORROSION-RESISTANT FULLY THREADED ROD END BOLT:12
- Mate:242: robotface-final:1 ↔ SetScrewLiteHub-1308-0016-0006:2
- Mate:244: robotface-final:1 ↔ StandoffM4-1501-0006-0420:1
- Mate:245: robotface-final:1 ↔ StandoffM4-1501-0006-0420:1
- Mate:246: robotface-final:1 ↔ StandoffM4-1501-0006-0420:2
- Mate:247: robotface-final:1 ↔ StandoffM4-1501-0006-0420:2
- Mate:248: robotface-final:1 ↔ StandoffM4-1501-0006-0340:1
- Mate:249: robotface-final:1 ↔ StandoffM4-1501-0006-0340:1
- Mate:250: robotface-final:1 ↔ StandoffM4-1501-0006-0340:2
- Mate:251: robotface-final:1 ↔ StandoffM4-1501-0006-0340:2
- [Mate]: HingedThreadedStandoffPart2:13 ↔ HingedThreadedStandoffPart1:6
- [Mate]: HingedThreadedStandoffPart2:13 ↔ HingedThreadedStandoffPart1:6
- Mate:254: robotface-final:1 ↔ HingedThreadedStandoffPart1:6
- Mate:255: robotface-final:1 ↔ HingedThreadedStandoffPart1:6
- Angle:47 (0 deg): robotface-final:1 ↔ HingedThreadedStandoffPart1:6
- Mate:256: HingedThreadedStandoffPart2:13 ↔ ShaftD6Female-632Female:5
- Mate:257: HingedThreadedStandoffPart2:13 ↔ ShaftD6Female-632Female:5
- [Mate]: UJoint6D-CenterDrive-4003-1006-1006:5 ↔ UJoint6D-Body-4003-1006-1006:10
- [Mate]: UJoint6D-CenterDrive-4003-1006-1006:5 ↔ UJoint6D-Body-4003-1006-1006:10
- [Mate]: UJoint6D-Body-4003-1006-1006:9 ↔ UJoint6D-CenterDrive-4003-1006-1006:5
- [Mate]: UJoint6D-Body-4003-1006-1006:9 ↔ UJoint6D-CenterDrive-4003-1006-1006:5
- [Mate]: UJoint6D-Body-4003-1006-1006:9 ↔ UJoint6D-Screw:19
- [Mate]: UJoint6D-Body-4003-1006-1006:9 ↔ UJoint6D-Screw:19
- [Mate]: UJoint6D-Body-4003-1006-1006:9 ↔ UJoint6D-Screw:21
- [Mate]: UJoint6D-Body-4003-1006-1006:9 ↔ UJoint6D-Screw:21
- [Mate]: UJoint6D-Body-4003-1006-1006:10 ↔ UJoint6D-Screw:20
- [Mate]: UJoint6D-Body-4003-1006-1006:10 ↔ UJoint6D-Screw:20
- [Mate]: UJoint6D-Body-4003-1006-1006:10 ↔ UJoint6D-Screw:22
- [Mate]: UJoint6D-Body-4003-1006-1006:10 ↔ UJoint6D-Screw:22
- [Mate]: ShaftD6-2100-0006-0250:3 ↔ UJoint6D-Body-4003-1006-1006:10
- [Angle] (0 deg): ShaftD6-2100-0006-0250:3 ↔ UJoint6D-Body-4003-1006-1006:10
- [Flush]: ShaftD6-2100-0006-0250:3 ↔ UJoint6D-Body-4003-1006-1006:10
- [Angle] (0 deg): UJoint6D-Body-4003-1006-1006:9 ↔ ShaftD6-Short-2101-0006-0020:5
- [Mate]: UJoint6D-Body-4003-1006-1006:9 ↔ ShaftD6-Short-2101-0006-0020:5
- [Flush]: UJoint6D-Body-4003-1006-1006:9 ↔ ShaftD6-Short-2101-0006-0020:5
- [Mate]: SetScrewLiteHub-1308-0016-0006:5 ↔ ShaftD6-Short-2101-0006-0020:5
- [Flush]: SetScrewLiteHub-1308-0016-0006:5 ↔ ShaftD6-Short-2101-0006-0020:5
- Mate:273: ShaftD6Female-632Female:5 ↔ ShaftD6-2100-0006-0250:3
- Angle:50 (0 deg): ShaftD6Female-632Female:5 ↔ ShaftD6-2100-0006-0250:3
- Mate:274: ShaftD6Female-632Female:5 ↔ ShaftD6-2100-0006-0250:3
- Mate:277: robotface-final:1 ↔ HeadEyeMount:1
- Mate:278: robotface-final:1 ↔ TongueMount:2
- Mate:281: TongueMount:2 ↔ SetScrewLiteHub-1308-0016-0006:1
- Mate:282: robotface-final:1 ↔ ClampingHub1301-0016-0012:1
- Mate:283: TongueMount:2 ↔ HingedThreadedStandoffPart2:6
- Mate:284: HingedThreadedStandoffPart2:1 ↔ TongueMount:2
- [Mate]: UJoint6D-CenterDrive-4003-1006-1006:6 ↔ UJoint6D-Body-4003-1006-1006:12
- [Mate]: UJoint6D-CenterDrive-4003-1006-1006:6 ↔ UJoint6D-Body-4003-1006-1006:12
- [Mate]: UJoint6D-Body-4003-1006-1006:11 ↔ UJoint6D-CenterDrive-4003-1006-1006:6
- [Mate]: UJoint6D-Body-4003-1006-1006:11 ↔ UJoint6D-CenterDrive-4003-1006-1006:6
- [Mate]: UJoint6D-Body-4003-1006-1006:11 ↔ UJoint6D-Screw:23
- [Mate]: UJoint6D-Body-4003-1006-1006:11 ↔ UJoint6D-Screw:23
- [Mate]: UJoint6D-Body-4003-1006-1006:11 ↔ UJoint6D-Screw:25
- [Mate]: UJoint6D-Body-4003-1006-1006:11 ↔ UJoint6D-Screw:25
- [Mate]: UJoint6D-Body-4003-1006-1006:12 ↔ UJoint6D-Screw:24
- [Mate]: UJoint6D-Body-4003-1006-1006:12 ↔ UJoint6D-Screw:24
- [Mate]: UJoint6D-Body-4003-1006-1006:12 ↔ UJoint6D-Screw:26
- [Mate]: UJoint6D-Body-4003-1006-1006:12 ↔ UJoint6D-Screw:26
- Angle:51 (0 deg): ShaftD6-Short-2101-0006-0020:1 ↔ UJoint6D-Body-4003-1006-1006:12
- Mate:297: ShaftD6-Short-2101-0006-0020:1 ↔ UJoint6D-Body-4003-1006-1006:12
- Flush:22: ShaftD6-Short-2101-0006-0020:1 ↔ UJoint6D-Body-4003-1006-1006:12
- Mate:298: ShaftD6-2100-0006-0250:1 ↔ UJoint6D-Body-4003-1006-1006:11
- Angle:52 (180 deg): ShaftD6-2100-0006-0250:1 ↔ UJoint6D-Body-4003-1006-1006:11
- Flush:23: ShaftD6-2100-0006-0250:1 ↔ UJoint6D-Body-4003-1006-1006:11
- Angle:53 (0 deg): SetScrewLiteHub-1308-0016-0006:1 ↔ UJoint6D-Body-4003-1006-1006:12
- Angle:54 (0 deg): ShaftD6-2100-0006-0250:1 ↔ HeadTongueMount:1
- Mate:299: LinearBearing-1612-0612-0035:1 ↔ ShaftD6-2100-0006-0250:1
- Mate:300: LinearBearing-1612-0612-0035:1 ↔ ClampingHub1301-0016-0012:1
- Flush:24: TongueMount:2 ↔ SetScrewLiteHub-1308-0016-0006:1
- Flush:25 (6 mm): LinearBearing-1612-0612-0035:1 ↔ ClampingHub1301-0016-0012:1
- [Mate]: UJoint6D-CenterDrive-4003-1006-1006:7 ↔ UJoint6D-Body-4003-1006-1006:14
- [Mate]: UJoint6D-CenterDrive-4003-1006-1006:7 ↔ UJoint6D-Body-4003-1006-1006:14
- [Mate]: UJoint6D-Body-4003-1006-1006:13 ↔ UJoint6D-CenterDrive-4003-1006-1006:7
- [Mate]: UJoint6D-Body-4003-1006-1006:13 ↔ UJoint6D-CenterDrive-4003-1006-1006:7
- [Mate]: UJoint6D-Body-4003-1006-1006:13 ↔ UJoint6D-Screw:28
- [Mate]: UJoint6D-Body-4003-1006-1006:13 ↔ UJoint6D-Screw:28
- [Mate]: UJoint6D-Body-4003-1006-1006:14 ↔ UJoint6D-Screw:27
- [Mate]: UJoint6D-Body-4003-1006-1006:14 ↔ UJoint6D-Screw:27
- [Mate]: UJoint6D-Body-4003-1006-1006:14 ↔ UJoint6D-Screw:29
- [Mate]: UJoint6D-Body-4003-1006-1006:14 ↔ UJoint6D-Screw:29
- Mate:311: ShaftD6-2100-0006-0250:1 ↔ UJoint6D-Body-4003-1006-1006:14
- Angle:55 (180 deg): ShaftD6-2100-0006-0250:1 ↔ UJoint6D-Body-4003-1006-1006:14
- Flush:26: ShaftD6-2100-0006-0250:1 ↔ UJoint6D-Body-4003-1006-1006:14
- Mate:312: ShaftD6-Short-2101-0006-0020:4 ↔ UJoint6D-Body-4003-1006-1006:13
- Angle:56 (180 deg): ShaftD6-Short-2101-0006-0020:4 ↔ UJoint6D-Body-4003-1006-1006:13
- Flush:27: ShaftD6-Short-2101-0006-0020:4 ↔ UJoint6D-Body-4003-1006-1006:13
- Mate:313: ShaftD6-Short-2101-0006-0020:4 ↔ SetScrewLiteHub-1308-0016-0006:6
- Angle:57 (0 deg): UJoint6D-Body-4003-1006-1006:13 ↔ SetScrewLiteHub-1308-0016-0006:6
- Flush:28: ShaftD6-Short-2101-0006-0020:4 ↔ SetScrewLiteHub-1308-0016-0006:6
- Mate:314: ArducamHat:1 ↔ M3-Standoff-30mm:1
- Mate:315: HeadEyeMount:1 ↔ M3-Standoff-30mm:1
- Mate:316: ArducamHat:1 ↔ M3-Standoff-30mm:1
- Mate:317: ArducamHat:1 ↔ M3-Standoff-30mm:2
- Mate:318: ArducamHat:1 ↔ M3-Standoff-30mm:2
- Mate:319: ArducamHat:1 ↔ M3-Standoff-30mm:3
- Mate:320: HeadEyeMount:1 ↔ M3-Standoff-30mm:3
- Mate:341: HeadEyeMount:1 ↔ M5-Standoff-32mm:1
- Mate:342: HeadMount:1 ↔ M5-Standoff-32mm:1
- Mate:343: HeadEyeMount:1 ↔ M5-Standoff-32mm:1
- Mate:344: HeadEyeMount:1 ↔ M5-Standoff-32mm:2
- Mate:345: HeadMount:1 ↔ M5-Standoff-32mm:2
- Mate:346: HeadMount:1 ↔ M5-Standoff-32mm:3
- Mate:347: HeadMount:1 ↔ M5-Standoff-32mm:4
- Mate:348: HeadEyeMount:1 ↔ M5-Standoff-32mm:4
- Mate:349: HeadEyeMount:1 ↔ M5-Standoff-32mm:3
- Mate:350: Arducam:2 ↔ HeadEyeMount:1
- Mate:351: Arducam:2 ↔ HeadEyeMount:1
- Mate:352: Arducam:2 ↔ M1-Standoff-20mm:1
- Mate:353: HeadEyeMount:1 ↔ M1-Standoff-20mm:1
- Mate:354: Arducam:2 ↔ M1-Standoff-20mm:2
- Mate:355: HeadEyeMount:1 ↔ M1-Standoff-20mm:2
- Mate:356: Arducam:2 ↔ M1-Standoff-20mm:3
- Mate:357: HeadEyeMount:1 ↔ M1-Standoff-20mm:3
- Mate:358: ArducamMirror:1 ↔ M1-Standoff-20mm:4
- Mate:359: HeadEyeMount:1 ↔ M1-Standoff-20mm:4
- Mate:360: HeadEyeMount:1 ↔ M1-Standoff-20mm:4
- Mate:361: ArducamMirror:1 ↔ M1-Standoff-20mm:5
- Mate:362: HeadEyeMount:1 ↔ M1-Standoff-20mm:5
- Mate:363: ArducamMirror:1 ↔ M1-Standoff-20mm:5
- Mate:364: Arducam:2 ↔ M1-Standoff-20mm:2
- Mate:365: HeadEyeMount:1 ↔ M1-Standoff-20mm:5
- Mate:366: ArducamMirror:1 ↔ M1-Standoff-20mm:6
- Mate:367: HeadEyeMount:1 ↔ M1-Standoff-20mm:6
- Mate:368: robotface-final:1 ↔ NoseInsideConnector:1
- Mate:369: robotface-final:1 ↔ NoseInsideConnector:1
- Angle:58 (0 deg): robotface-final:1 ↔ NoseInsideConnector:1
- Mate:370: SetScrewLiteHub-1308-0016-0006:2 ↔ NoseInsideConnector:1
- Mate:371: SetScrewLiteHub-1308-0016-0006:2 ↔ NoseInsideConnector:1
- Mate:372: Part2^3mm U-Joint:1 ↔ Part1^3mm U-Joint:1
- Mate:373 (0.15 mm): Part2^3mm U-Joint:1 ↔ Part1^3mm U-Joint:1
- Mate:374: Part2^3mm U-Joint:1 ↔ Part1^3mm U-Joint:2
- Mate:375 (0.15 mm): Part2^3mm U-Joint:1 ↔ Part1^3mm U-Joint:2
- [Mate]: Part2^3mm U-Joint:2 ↔ Part1^3mm U-Joint:3
- [Mate] (0.15 mm): Part2^3mm U-Joint:2 ↔ Part1^3mm U-Joint:3
- [Mate]: Part2^3mm U-Joint:2 ↔ Part1^3mm U-Joint:4
- [Mate] (0.15 mm): Part2^3mm U-Joint:2 ↔ Part1^3mm U-Joint:4
- Mate:380: robotface-final:1 ↔ Part1^3mm U-Joint:2
- Mate:381: robotface-final:1 ↔ Part1^3mm U-Joint:2
- Mate:382: robotface-final:1 ↔ Part1^3mm U-Joint:4
- Mate:383: robotface-final:1 ↔ Part1^3mm U-Joint:4
- Mate:384: NoseInsideConnector:1 ↔ Part1^3mm U-Joint:3
- Mate:385: NoseInsideConnector:1 ↔ Part1^3mm U-Joint:1
- Mate:386: robotface-final:1 ↔ NoseCover:1
- Mate:387: robotface-final:1 ↔ NoseCover:1
- Flush:29: NoseCover:1 ↔ NoseCoverSmall:1
- Mate:388 (10 mm): NoseCover:1 ↔ NoseCoverSmall:1
- Mate:389: robotface-final:1 ↔ NoseCoverSmall:1
- Mate:390: Arducam:2 ↔ IRLed-FY-4006:2
- Mate:391: ArducamMirror:1 ↔ IRLed-FY-4006:1
- Mate:392: HeadMount:1 ↔ BackEyeMountLeft:1
- Mate:393: HeadMount:1 ↔ BackEyeMountLeft:1
- Mate:394: HeadMount:1 ↔ BackEyeMountLeft:1
- Mate:395: IRLed-FY-4006:3 ↔ BackEyeMountLeft:1
- Mate:396: IRLed-FY-4006:3 ↔ BackEyeMountLeft:1
- Mate:397: IRLed-FY-4006:3 ↔ BackEyeMountLeft:1
- Mate:398: HeadMount:1 ↔ BackEyeMountRight:1
- Mate:399: HeadMount:1 ↔ BackEyeMountRight:1
- Mate:400: HeadMount:1 ↔ BackEyeMountRight:1
- Mate:401: BackEyeMountRight:1 ↔ IRLed-FY-4006:4
- Mate:402: BackEyeMountRight:1 ↔ IRLed-FY-4006:4
- Mate:403: BackEyeMountRight:1 ↔ IRLed-FY-4006:4
- Mate:404: robotface-final:1 ↔ ShaftClamp6-6058N14:1
- Mate:405: robotface-final:1 ↔ ShaftClamp6-6058N14:1
- [Mate]: robotface-final:1 ↔ ShaftD6-2100-0006-0200:1
- [Mate]: robotface-final:1 ↔ ShaftD6-2100-0006-0200:1
- [Mate]: robotface-final:1 ↔ ShaftD6-2100-0006-0200:2
- [Mate]: ShaftD6-2100-0006-0200:2 ↔ ShaftClamp6-6058N14:2
- [Flush]: robotface-final:1 ↔ ShaftD6-2100-0006-0200:2
- [Mate]: ShaftD6-2100-0006-0200:3 ↔ ShaftClamp6-6058N14:3
- [Mate]: robotface-final:1 ↔ ShaftD6-2100-0006-0200:3
- [Flush]: robotface-final:1 ↔ ShaftD6-2100-0006-0200:3
- Mate:414: robotface-final:1 ↔ ShaftClamp6-6058N14:4
- Mate:415: robotface-final:1 ↔ ShaftClamp6-6058N14:4
- Mate:416: robotface-final:1 ↔ ShaftClamp6-6058N14:5
- Mate:417: robotface-final:1 ↔ ShaftClamp6-6058N14:5
- Mate:418: robotface-final:1 ↔ ShaftClamp6-6058N14:6
- Mate:419: robotface-final:1 ↔ ShaftClamp6-6058N14:6
- [Mate]: ShaftD6-2100-0006-0200:4 ↔ ShaftClamp6-6058N14:6
- [Mate]: robotface-final:1 ↔ ShaftD6-2100-0006-0200:4
- [Mate]: ShaftD6-2100-0006-0200:5 ↔ ShaftClamp6-6058N14:7
- [Mate]: robotface-final:1 ↔ ShaftD6-2100-0006-0200:5
- [Flush]: robotface-final:1 ↔ ShaftD6-2100-0006-0200:5
- [Mate]: ShaftD6-2100-0006-0200:6 ↔ ShaftClamp6-6058N14:8
- [Mate]: robotface-final:1 ↔ ShaftD6-2100-0006-0200:6
- [Flush]: robotface-final:1 ↔ ShaftD6-2100-0006-0200:6
- Mate:428: MuzzleHeadMount:1 ↔ MuzzleHeadConnector:1
- Mate:429: MuzzleHeadMount:1 ↔ MuzzleHeadConnector:1
- Mate:430: MuzzleHeadMount:1 ↔ MuzzleHeadConnector:1
- Mate:431: HeadTongueMount:1 ↔ MuzzleHeadConnector:1
- Mate:432: ShaftD6-2100-0006-0200:1 ↔ ShaftClamp6-6058N14:9
- Mate:434: MuzzleHeadMount:1 ↔ ShaftClamp6-6058N14:9
- Mate:435: MuzzleHeadMount:1 ↔ ShaftClamp6-6058N14:10
- Mate:436: ShaftD6-2100-0006-0200:1 ↔ ShaftClamp6-6058N14:10
- Mate:437: ShaftD6-2100-0006-0200:4 ↔ ShaftClamp6-6058N14:12
- Mate:438: MuzzleHeadMount:1 ↔ ShaftClamp6-6058N14:12
- Mate:439: ShaftD6-2100-0006-0200:4 ↔ ShaftClamp6-6058N14:13
- Mate:440: MuzzleHeadMount:1 ↔ ShaftClamp6-6058N14:13
- Mate:441: ShaftD6-2100-0006-0200:2 ↔ ShaftClamp6-6058N14:14
- Mate:442: MuzzleHeadMount:1 ↔ ShaftClamp6-6058N14:14
- Mate:443: ShaftD6-2100-0006-0200:2 ↔ ShaftClamp6-6058N14:15
- Mate:444: MuzzleHeadMount:1 ↔ ShaftClamp6-6058N14:15
- Mate:445: ShaftD6-2100-0006-0200:3 ↔ ShaftClamp6-6058N14:16
- Mate:446: MuzzleHeadMount:1 ↔ ShaftClamp6-6058N14:16
- Mate:447: ShaftD6-2100-0006-0200:3 ↔ ShaftClamp6-6058N14:17
- Mate:448: MuzzleHeadMount:1 ↔ ShaftClamp6-6058N14:17
- Mate:449: ShaftD6-2100-0006-0200:5 ↔ ShaftClamp6-6058N14:18
- Mate:450: MuzzleHeadMount:1 ↔ ShaftClamp6-6058N14:18
- Mate:451: ShaftD6-2100-0006-0200:5 ↔ ShaftClamp6-6058N14:19
- Mate:452: MuzzleHeadMount:1 ↔ ShaftClamp6-6058N14:19
- Mate:453: ShaftD6-2100-0006-0200:6 ↔ ShaftClamp6-6058N14:20
- Mate:454: MuzzleHeadMount:1 ↔ ShaftClamp6-6058N14:20
- Mate:455: ShaftD6-2100-0006-0200:6 ↔ ShaftClamp6-6058N14:21
- Mate:456: MuzzleHeadMount:1 ↔ ShaftClamp6-6058N14:21
- Mate:458: ShaftD6-2100-0006-0200:2 ↔ BackSideConnector:1
- Mate:461: VacuumTubeHolder:2 ↔ BackSideConnector:1
- Mate:462: VacuumTubeHolder:2 ↔ BackSideConnector:1
- Mate:463: robotface-final:1 ↔ BackSideConnector:1
- Mate:464: ShaftClamp6-6058N14:2 ↔ BackSideConnector:1
- Mate:465: robotface-final:1 ↔ BackSideConnector:2
- Mate:466: ShaftD6-2100-0006-0200:3 ↔ BackSideConnector:2
- Mate:467: VacuumTubeHolder:1 ↔ BackSideConnector:2
- Mate:468: VacuumTubeHolder:1 ↔ BackSideConnector:2
- Mate:469: robotface-final:1 ↔ BackSideConnector:3
- Mate:470: ShaftD6-2100-0006-0200:6 ↔ BackSideConnector:3
- Mate:471: ShaftClamp6-6058N14:8 ↔ BackSideConnector:3
- Mate:472: VacuumTubeHolder:4 ↔ BackSideConnector:3
- Mate:473: VacuumTubeHolder:4 ↔ BackSideConnector:3
- Mate:474: robotface-final:1 ↔ BackSideConnector:4
- Mate:475: ShaftD6-2100-0006-0200:5 ↔ BackSideConnector:4
- Mate:476: ShaftClamp6-6058N14:7 ↔ BackSideConnector:4
- Mate:477: VacuumTubeHolder:3 ↔ BackSideConnector:4
- Mate:478: VacuumTubeHolder:3 ↔ BackSideConnector:4
## Named parameters: d60_d58 = 0 mm, d61_d59 = 0 mm, d275_d245_d146 = 0 mm, d276_d246_d147 = 0 mm, d277_d247_d148 = 0 mm, d278_d248_d149 = 0 mm, d279_d249_d150 = 0 mm, d280_d250_d151 = 0 mm, d281_d251_d152 = 0 mm, d282_d252_d153 = 0 mm, d283_d253_d154 = 0 mm, d284_d254_d155 = 0 mm, d285_d255_d156 = 0 mm, d286_d256_d157 = 0 mm, d298_d245_d146 = 0 mm, d299_d246_d147 = 0 mm, d300_d247_d148 = 0 mm, d301_d248_d149 = 0 mm, d302_d249_d150 = 0 mm, d303_d250_d151 = 0 mm, d304_d251_d152 = 0 mm, d305_d252_d153 = 0 mm, d306_d253_d154 = 0 mm, d307_d254_d155 = 0 mm, d308_d255_d156 = 0 mm, d309_d256_d157 = 0 mm, d433_d427 = 0 mm, d434_d428 = 0 mm, d435_d429 = 0 mm, d436_d431 = 0 mm, d440_d427 = 0 mm, d441_d428 = 0 mm, d442_d429 = 0 mm, d443_d431 = 0 mm, d447_d440_d427 = 0 mm, d448_d441_d428 = 0 mm, d449_d442_d429 = 0 mm, d450_d443_d431 = 0 mm, d466_d58 = 0 mm, d467_d59 = 0 mm, d474_d352 = 0 deg, d475_d353 = 0 mm, d476_d354 = 0 mm, d477_d355 = 0 mm, d478_d356 = 0 mm, d479_d257 = 0 mm, d480_d258 = 0 deg, d481_d259 = 0 mm, d482_d245_d146 = 0 mm, d483_d246_d147 = 0 mm, d484_d247_d148 = 0 mm, d485_d248_d149 = 0 mm, d486_d249_d150 = 0 mm, d487_d250_d151 = 0 mm, d488_d251_d152 = 0 mm, d489_d252_d153 = 0 mm, d490_d253_d154 = 0 mm, d491_d254_d155 = 0 mm, d492_d255_d156 = 0 mm, d493_d256_d157 = 0 mm, d512_d245_d146 = 0 mm, d513_d246_d147 = 0 mm, d514_d247_d148 = 0 mm, d515_d248_d149 = 0 mm, d516_d249_d150 = 0 mm, d517_d250_d151 = 0 mm, d518_d251_d152 = 0 mm, d519_d252_d153 = 0 mm, d520_d253_d154 = 0 mm, d521_d254_d155 = 0 mm, d522_d255_d156 = 0 mm, d523_d256_d157 = 0 mm, d539_d298_d245_d146 = 0 mm, d540_d299_d246_d147 = 0 mm, d541_d300_d247_d148 = 0 mm, d542_d301_d248_d149 = 0 mm, d543_d304_d251_d152 = 0 mm, d544_d305_d252_d153 = 0 mm, d545_d306_d253_d154 = 0 mm, d546_d307_d254_d155 = 0 mm, d547_d308_d255_d156 = 0 mm, d548_d309_d256_d157 = 0 mm, d629_d625 = 0 mm, d630_d626 = 0.15 mm, d631_d627 = 0 mm, d632_d628 = 0.15 mm, d678_d675 = 0 mm, d692_d678_d675 = 0 mm, d696_d692_d678_d675 = 0 mm
